# Autodesk Inventor assembly: Erasmus3
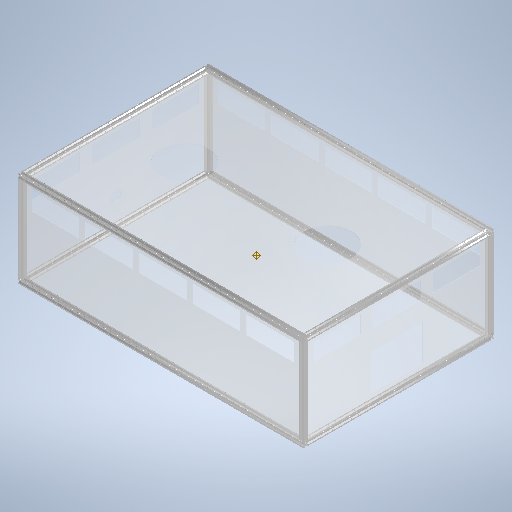
[picture p0: Inventor's stored thumbnail of the model, 512x512]
Saved by Autodesk Inventor 2025.1 (Build 291241000, 241)
## iProperties
Created: 2024-09-09
Part Number: Erasmus3
Document SubType Name: Assembly
Designer: joser
Author: joser
## Documents named in this file (9)
- C:\Users\joser\Documents\PUCP SSD\PUCP\Investigacion\Erasmus\Diseño pruebas\Erasmus3.iam
- C:\Users\joser\Documents\PUCP SSD\PUCP\Investigacion\Erasmus\Diseño pruebas\v-slot_L.ipt
- C:\Users\joser\Documents\PUCP SSD\PUCP\Investigacion\Erasmus\Diseño pruebas\v-slot_W.ipt
- C:\Users\joser\Documents\PUCP SSD\PUCP\Investigacion\Erasmus\Diseño pruebas\Base.ipt
- C:\Users\joser\Documents\PUCP SSD\PUCP\Investigacion\Erasmus\Diseño pruebas\v-slot_H.ipt
- C:\Users\joser\Documents\PUCP SSD\PUCP\Investigacion\Erasmus\Diseño pruebas\Lado.ipt
- C:\Users\joser\Documents\PUCP SSD\PUCP\Investigacion\Erasmus\Diseño pruebas\Anterior.ipt
- C:\Users\joser\Documents\PUCP SSD\PUCP\Investigacion\Erasmus\Diseño pruebas\Posterior.ipt
- C:\Users\joser\Documents\PUCP SSD\PUCP\Investigacion\Erasmus\Diseño pruebas\Tapa.ipt
## Components (18 placed, 8 different names)
1. v-slot_L:1 — Mate:1, Flush:1, Flush:2, Mate:2, Flush:3, Flush:4, Mate:7, Flush:8, Mate:8, Mate:9, Flush:9, Flush:10, Mate:10, Flush:11, Flush:12
2. v-slot_L:2 — Mate:3, Flush:5, Flush:6, Mate:11, Flush:13, Flush:14, Mate:12, Flush:15, Flush:16, Mate:14
3. v-slot_L:3 — Mate:13, Flush:20, Flush:21, Mate:16, Flush:26, Flush:27, Mate:17, Flush:28, Flush:29
4. v-slot_L:4 — Mate:15, Flush:24, Flush:25
5. v-slot_W:1 — Mate:1, Flush:1, Flush:2, Mate:3, Flush:5, Flush:6
6. v-slot_W:2 — Mate:2, Flush:3, Flush:4
7. Base:1 — Mate:5, Flush:7, Mate:6, Mate:7, Flush:8, Mate:8
8. v-slot_H:1 — Mate:9, Flush:9, Flush:10, Flush:17, Flush:18, Mate:13
9. v-slot_H:2 — Mate:11, Flush:13, Flush:14, Flush:23
10. v-slot_H:3 — Mate:10, Flush:11, Flush:12, Flush:20, Flush:21
11. v-slot_H:4 — Mate:12, Flush:15, Flush:16, Mate:15, Flush:24, Flush:25
12. v-slot_W:3 — Mate:16, Flush:26, Flush:27, Flush:30
13. v-slot_W:4 — Mate:17, Flush:28, Flush:29, Flush:35, Flush:38
14. Lado:1 — Flush:17, Flush:18, Flush:19
15. Lado:2 — Mate:14, Flush:22, Flush:23
16. Anterior:1 — Flush:30, Flush:31, Flush:32
17. Posterior:1 — Flush:33, Flush:34, Flush:35
18. Tapa:1 — Flush:36, Flush:37, Flush:38
## Relationships (54: Flush 38, Mate 16)
- Mate:1: v-slot_L:1 ↔ v-slot_W:1
- Flush:1: v-slot_L:1 ↔ v-slot_W:1
- Flush:2: v-slot_L:1 ↔ v-slot_W:1
- Mate:2: v-slot_L:1 ↔ v-slot_W:2
- Flush:3: v-slot_L:1 ↔ v-slot_W:2
- Flush:4: v-slot_L:1 ↔ v-slot_W:2
- Mate:3: v-slot_L:2 ↔ v-slot_W:1
- Flush:5: v-slot_L:2 ↔ v-slot_W:1
- Flush:6: v-slot_L:2 ↔ v-slot_W:1
- Mate:5: Base:1
- Flush:7: Base:1
- Mate:6 (-190 mm): Base:1
- Mate:7: v-slot_L:1 ↔ Base:1
- Flush:8 (600 mm): v-slot_L:1 ↔ Base:1
- Mate:8 (-400 mm): v-slot_L:1 ↔ Base:1
- Mate:9: v-slot_L:1 ↔ v-slot_H:1
- Flush:9: v-slot_L:1 ↔ v-slot_H:1
- Flush:10: v-slot_L:1 ↔ v-slot_H:1
- Mate:10: v-slot_L:1 ↔ v-slot_H:3
- Flush:11: v-slot_L:1 ↔ v-slot_H:3
- Flush:12: v-slot_L:1 ↔ v-slot_H:3
- Mate:11: v-slot_L:2 ↔ v-slot_H:2
- Flush:13: v-slot_L:2 ↔ v-slot_H:2
- Flush:14: v-slot_L:2 ↔ v-slot_H:2
- Mate:12: v-slot_L:2 ↔ v-slot_H:4
- Flush:15: v-slot_L:2 ↔ v-slot_H:4
- Flush:16: v-slot_L:2 ↔ v-slot_H:4
- Flush:17: v-slot_H:1 ↔ Lado:1
- Flush:18 (-590 mm): v-slot_H:1 ↔ Lado:1
- Flush:19: Lado:1
- Mate:13: v-slot_L:3 ↔ v-slot_H:1
- Flush:20: v-slot_L:3 ↔ v-slot_H:3
- Flush:21: v-slot_L:3 ↔ v-slot_H:3
- Mate:14: v-slot_L:2 ↔ Lado:2
- Flush:22: Lado:2
- Flush:23 (590 mm): v-slot_H:2 ↔ Lado:2
- Mate:15: v-slot_L:4 ↔ v-slot_H:4
- Flush:24: v-slot_L:4 ↔ v-slot_H:4
- Flush:25: v-slot_L:4 ↔ v-slot_H:4
- Mate:16: v-slot_L:3 ↔ v-slot_W:3
- Flush:26: v-slot_L:3 ↔ v-slot_W:3
- Flush:27: v-slot_L:3 ↔ v-slot_W:3
- Mate:17: v-slot_L:3 ↔ v-slot_W:4
- Flush:28: v-slot_L:3 ↔ v-slot_W:4
- Flush:29: v-slot_L:3 ↔ v-slot_W:4
- Flush:30: v-slot_W:3 ↔ Anterior:1
- Flush:31: Anterior:1
- Flush:32: Anterior:1
- Flush:33: Posterior:1
- Flush:34: Posterior:1
- Flush:35: v-slot_W:4 ↔ Posterior:1
- Flush:36: Tapa:1
- Flush:37: Tapa:1
- Flush:38: v-slot_W:4 ↔ Tapa:1
